# Autodesk Inventor assembly: arl2-16-70
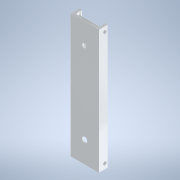
[picture p0: Inventor's stored thumbnail of the model, 180x180]
Saved by Autodesk Inventor 2021 (Build 250183000, 183)
## iProperties
Created: 2014-06-16
Part Number: arl2-16-70
Description: STEP AP214
Document SubType Name: Assembly
Designer: Ryohei
Sending System: SolidWorks 2013
Preprocessor: SwSTEP 2.0
Title: arl2-16-70.step
Revision Number: ANY
## Documents named in this file (3)
- C:\Users\Hagihara Yuya\Documents\GrabCAD\NHK2021\BasicParts\よく使う部品（萩原）\SlideRail\arl2-16-70\arl2-16-70.iam
- C:\Users\Hagihara Yuya\Documents\GrabCAD\NHK2021\BasicParts\よく使う部品（萩原）\SlideRail\arl2-16-70\arl2-16-70-01.ipt
- C:\Users\Hagihara Yuya\Documents\GrabCAD\NHK2021\BasicParts\よく使う部品（萩原）\SlideRail\arl2-16-70\arl2-16-70-02.ipt
## Components (2 placed, 2 different names)
1. arl2-16-70-01_1 — スライダ:1
2. arl2-16-70-02_2 — スライダ:1
## Relationships (1: TranslationJoint 1)
- スライダ:1 [TranslationJoint] (-6 mm): arl2-16-70-01_1 ↔ arl2-16-70-02_2
